# Autodesk Inventor assembly: LAP_RAP
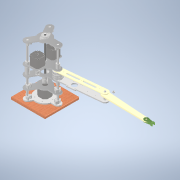
[picture p0: Inventor's stored thumbnail of the model, 180x180]
Saved by Autodesk Inventor 2022 (Build 260153000, 153)
## iProperties
Created: 2022-11-10
Part Number: LAP_RAP
Document SubType Name: Assembly
Designer: nguye
Author: nguye
## Documents named in this file (25)
- C:\Users\nguye\Documents\Inventor\ROBOT\LAP_RAP.iam
- C:\Users\nguye\Documents\Inventor\ROBOT\De_Duoi.ipt
- C:\Users\nguye\Documents\Inventor\ROBOT\De_Go.ipt
- C:\Users\nguye\Documents\Inventor\ROBOT\De_Tren.ipt
- C:\Users\nguye\Documents\Inventor\ROBOT\Truc_8mm.ipt
- C:\Users\nguye\Documents\Inventor\ROBOT\DAI_OC.ipt
- C:\Users\nguye\Documents\Inventor\ROBOT\KN_5_8.ipt
- C:\Users\nguye\Documents\Inventor\ROBOT\O_Do_Lan.ipt
- C:\Users\nguye\Documents\Inventor\ROBOT\De_Tren_Cung.ipt
- C:\Users\nguye\Documents\Inventor\ROBOT\Vit_me.ipt
- C:\Users\nguye\Documents\Inventor\ROBOT\De_2.ipt
- C:\Users\nguye\Documents\Inventor\ROBOT\Canh_Tay_1.ipt
- C:\Users\nguye\Documents\Inventor\ROBOT\Canh_Tay_2.ipt
- C:\Users\nguye\Documents\Inventor\ROBOT\Stepper.ipt
- C:\Users\nguye\Documents\Inventor\ROBOT\Con_Truot.ipt
- C:\Users\nguye\Documents\Inventor\ROBOT\Kep_Truc.ipt
- C:\Users\nguye\Documents\Inventor\ROBOT\Pully_Nho.ipt
- C:\Users\nguye\Documents\Inventor\ROBOT\Truc_5_mm.ipt
- C:\Users\nguye\Documents\Inventor\ROBOT\O_lan_5mm.ipt
- C:\Users\nguye\Documents\Inventor\ROBOT\KEP_BUT.ipt
- C:\Users\nguye\Documents\Inventor\ROBOT\Lot_Truot.ipt
- C:\Users\nguye\Documents\Inventor\ROBOT\De_Mica.ipt
- C:\Users\nguye\Documents\Inventor\ROBOT\Puly_60_double - Copy.ipt
- C:\Users\nguye\Documents\Inventor\ROBOT\Puly_60_teeth.ipt
- C:\Users\nguye\Documents\Inventor\ROBOT\Tess.ipt
## Components (45 placed, 24 different names)
1. De_0 — Mate:28, Mate:29, Mate:44, Mate:61, Mate:62, Mate:64, Mate:65, Mate:67, Mate:68
2. De_Go:1 — Mate:1, Mate:2, Mate:3, Angle:5, Mate:72, Mate:74, Mate:76, Mate:126, Flush:15, Flush:16, Flush:17
3. De_2 — Mate:9, Mate:10, Mate:15, Mate:16, Mate:34, Mate:45, Angle:6, Mate:46, Mate:47, Angle:7, Mate:48, Flush:8, Flush:9, Flush:10, Mate:121, Mate:123
4. Truc_8mm:1 — Mate:2, Mate:10, Flush:4, Mate:31, Mate:49, Mate:50, Mate:66, Mate:71, Mate:80, Mate:120, Mate:125, Flush:17
5. Truc_8mm:2 — Mate:1, Mate:21, Mate:28, Mate:32, Mate:57, Mate:60, Mate:69, Mate:81, Mate:124, Flush:15, Mate:132, Mate:133, Mate:136
6. Truc_8mm:3 — Mate:3, Mate:9, Mate:29, Mate:30, Mate:51, Mate:54, Mate:63, Mate:70, Mate:78, Mate:79, Mate:122, Flush:16
7. DAI_OC:1 — Mate:15, Mate:16
8. KN_5_8:1 — Mate:27, Mate:40, Mate:41, Mate:42
9. O_Do_Lan:1 — Mate:23, Mate:24, Mate:25, Mate:26
10. De_3 — Mate:21, Mate:23, Mate:24, Mate:25, Flush:4, Mate:51, Mate:52, Mate:53, Mate:55, Mate:56, Mate:58, Mate:59
11. Vit_me:1 — Mate:26, Mate:27, Mate:42
12. De_1 — Mate:30, Mate:31, Flush:6, Flush:7, Mate:82, Flush:11, Mate:138
13. Canh_Tay_1:2 — Mate:32, Mate:34, Mate:99, Mate:103, Flush:12, Flush:13, Mate:108, Mate:134
14. Canh_Tay_2:1 — Mate:108, Mate:110, Angle:9, Mate:118, Mate:119, Angle:10
15. Stepper:4 — Mate:47, Angle:7, Mate:48, Mate:131
16. Stepper:5 — Mate:40, Mate:41, Angle:5, Mate:44, Mate:130
17. Stepper:6 — Mate:45, Angle:6, Mate:46, Mate:83
18. Con_Truot:1 — Mate:49, Flush:9
19. Con_Truot:2 — Mate:79, Flush:6
20. Con_Truot:3 — Flush:10, Mate:81
21. Con_Truot:4 — Mate:78, Flush:8
22. Con_Truot:5 — Mate:80, Flush:7
23. Kep_Truc:1 — Mate:63, Mate:64, Mate:65
24. Kep_Truc:2 — Mate:54, Mate:55, Mate:56
25. Kep_Truc:3 — Mate:60, Mate:61, Mate:62
26. Kep_Truc:4 — Mate:50, Mate:52, Mate:53
27. Kep_Truc:5 — Mate:57, Mate:58, Mate:59
28. Kep_Truc:6 — Mate:66, Mate:67, Mate:68
29. Kep_Truc:7 — Mate:70, Mate:72, Mate:129
30. Kep_Truc:8 — Mate:69, Mate:74, Mate:128
31. Kep_Truc:9 — Mate:71, Mate:76, Mate:127
32. Con_Truot:6 — Mate:82, Flush:11
33. Pully_Nho:1 — Mate:83
34. Truc_5_mm:1 — Mate:99, Flush:13, Mate:109, Mate:137
35. O_lan_5mm:1 — Mate:103, Flush:12
36. O_lan_5mm:2
37. Pully_Nho:3 — Mate:131
38. Pully_Nho:4 — Mate:109, Mate:110, Angle:9
39. KEP_BUT:1 — Mate:118, Mate:119, Angle:10
40. Lot_Truot:1 — Mate:120, Mate:121
41. Lot_Truot:2 — Mate:122, Mate:123
42. De_Mica:2 — Mate:124, Mate:125, Mate:126, Mate:127, Mate:128, Mate:129, Mate:130
43. Puly_60_double - Copy:1 — Mate:132, Mate:135, Mate:139
44. Puly_60_teeth:1 — Mate:133, Mate:134, Mate:135
45. Tess:1 — Mate:136, Mate:137, Mate:138, Mate:139
## Relationships (103: Mate 86, Flush 12, Angle 5)
- Mate:1: De_Go:1 ↔ Truc_8mm:2
- Mate:2: De_Go:1 ↔ Truc_8mm:1
- Mate:3: De_Go:1 ↔ Truc_8mm:3
- Mate:9: De_2 ↔ Truc_8mm:3
- Mate:10: De_2 ↔ Truc_8mm:1
- Mate:15: De_2 ↔ DAI_OC:1
- Mate:16: De_2 ↔ DAI_OC:1
- Mate:21: Truc_8mm:2 ↔ De_3
- Mate:23: O_Do_Lan:1 ↔ De_3
- Mate:24: O_Do_Lan:1 ↔ De_3
- Mate:25: O_Do_Lan:1 ↔ De_3
- Mate:26: O_Do_Lan:1 ↔ Vit_me:1
- Mate:27: KN_5_8:1 ↔ Vit_me:1
- Flush:4: Truc_8mm:1 ↔ De_3
- Mate:28: De_0 ↔ Truc_8mm:2
- Mate:29: De_0 ↔ Truc_8mm:3
- Mate:30: Truc_8mm:3 ↔ De_1
- Mate:31: Truc_8mm:1 ↔ De_1
- Mate:32: Truc_8mm:2 ↔ Canh_Tay_1:2
- Mate:34: De_2 ↔ Canh_Tay_1:2
- Mate:40: KN_5_8:1 ↔ Stepper:5
- Mate:41: KN_5_8:1 ↔ Stepper:5
- Mate:42: KN_5_8:1 ↔ Vit_me:1
- Angle:5 (0 deg): De_Go:1 ↔ Stepper:5
- Mate:44: De_0 ↔ Stepper:5
- Mate:45: De_2 ↔ Stepper:6
- Angle:6 (0 deg): De_2 ↔ Stepper:6
- Mate:46: De_2 ↔ Stepper:6
- Mate:47: De_2 ↔ Stepper:4
- Angle:7 (0 deg): De_2 ↔ Stepper:4
- Mate:48: De_2 ↔ Stepper:4
- Mate:49: Truc_8mm:1 ↔ Con_Truot:1
- Mate:50: Truc_8mm:1 ↔ Kep_Truc:4
- Mate:51: Truc_8mm:3 ↔ De_3
- Mate:52: De_3 ↔ Kep_Truc:4
- Mate:53: De_3 ↔ Kep_Truc:4
- Mate:54: Truc_8mm:3 ↔ Kep_Truc:2
- Mate:55: De_3 ↔ Kep_Truc:2
- Mate:56: De_3 ↔ Kep_Truc:2
- Mate:57: Truc_8mm:2 ↔ Kep_Truc:5
- Mate:58: De_3 ↔ Kep_Truc:5
- Mate:59: De_3 ↔ Kep_Truc:5
- Mate:60: Truc_8mm:2 ↔ Kep_Truc:3
- Mate:61: De_0 ↔ Kep_Truc:3
- Mate:62: De_0 ↔ Kep_Truc:3
- Mate:63: Truc_8mm:3 ↔ Kep_Truc:1
- Mate:64: De_0 ↔ Kep_Truc:1
- Mate:65: De_0 ↔ Kep_Truc:1
- Mate:66: Truc_8mm:1 ↔ Kep_Truc:6
- Mate:67: De_0 ↔ Kep_Truc:6
- Mate:68: De_0 ↔ Kep_Truc:6
- Mate:69: Truc_8mm:2 ↔ Kep_Truc:8
- Mate:70: Truc_8mm:3 ↔ Kep_Truc:7
- Mate:71: Truc_8mm:1 ↔ Kep_Truc:9
- Mate:72: De_Go:1 ↔ Kep_Truc:7
- Mate:74: De_Go:1 ↔ Kep_Truc:8
- Mate:76: De_Go:1 ↔ Kep_Truc:9
- Mate:78: Truc_8mm:3 ↔ Con_Truot:4
- Mate:79: Truc_8mm:3 ↔ Con_Truot:2
- Mate:80: Truc_8mm:1 ↔ Con_Truot:5
- Flush:6 (-10 mm): De_1 ↔ Con_Truot:2
- Flush:7 (-10 mm): De_1 ↔ Con_Truot:5
- Flush:8 (-10 mm): De_2 ↔ Con_Truot:4
- Flush:9 (-10 mm): De_2 ↔ Con_Truot:1
- Flush:10: De_2 ↔ Con_Truot:3
- Mate:81: Truc_8mm:2 ↔ Con_Truot:3
- Mate:82: De_1 ↔ Con_Truot:6
- Flush:11: De_1 ↔ Con_Truot:6
- Mate:83: Stepper:6 ↔ Pully_Nho:1
- Mate:99: Canh_Tay_1:2 ↔ Truc_5_mm:1
- Mate:103: Canh_Tay_1:2 ↔ O_lan_5mm:1
- Flush:12: Canh_Tay_1:2 ↔ O_lan_5mm:1
- Flush:13 (-4 mm): Canh_Tay_1:2 ↔ Truc_5_mm:1
- Mate:108 (5 mm): Canh_Tay_1:2 ↔ Canh_Tay_2:1
- Mate:109: Truc_5_mm:1 ↔ Pully_Nho:4
- Mate:110: Canh_Tay_2:1 ↔ Pully_Nho:4
- Angle:9 (0 deg): Canh_Tay_2:1 ↔ Pully_Nho:4
- Mate:118: Canh_Tay_2:1 ↔ KEP_BUT:1
- Mate:119: Canh_Tay_2:1 ↔ KEP_BUT:1
- Angle:10 (180 deg): Canh_Tay_2:1 ↔ KEP_BUT:1
- Mate:120: Truc_8mm:1 ↔ Lot_Truot:1
- Mate:121: De_2 ↔ Lot_Truot:1
- Mate:122: Truc_8mm:3 ↔ Lot_Truot:2
- Mate:123: De_2 ↔ Lot_Truot:2
- Mate:124: Truc_8mm:2 ↔ De_Mica:2
- Mate:125: Truc_8mm:1 ↔ De_Mica:2
- Mate:126: De_Go:1 ↔ De_Mica:2
- Flush:15: De_Go:1 ↔ Truc_8mm:2
- Flush:16: De_Go:1 ↔ Truc_8mm:3
- Flush:17: De_Go:1 ↔ Truc_8mm:1
- Mate:127: Kep_Truc:9 ↔ De_Mica:2
- Mate:128: Kep_Truc:8 ↔ De_Mica:2
- Mate:129: Kep_Truc:7 ↔ De_Mica:2
- Mate:130: Stepper:5 ↔ De_Mica:2
- Mate:131: Stepper:4 ↔ Pully_Nho:3
- Mate:132: Truc_8mm:2 ↔ Puly_60_double - Copy:1
- Mate:133: Truc_8mm:2 ↔ Puly_60_teeth:1
- Mate:134: Canh_Tay_1:2 ↔ Puly_60_teeth:1
- Mate:135 (1 mm): Puly_60_double - Copy:1 ↔ Puly_60_teeth:1
- Mate:136: Truc_8mm:2 ↔ Tess:1
- Mate:137: Truc_5_mm:1 ↔ Tess:1
- Mate:138: De_1 ↔ Tess:1
- Mate:139: Puly_60_double - Copy:1 ↔ Tess:1
